# Autodesk Inventor assembly: _VK_Indexier-Station
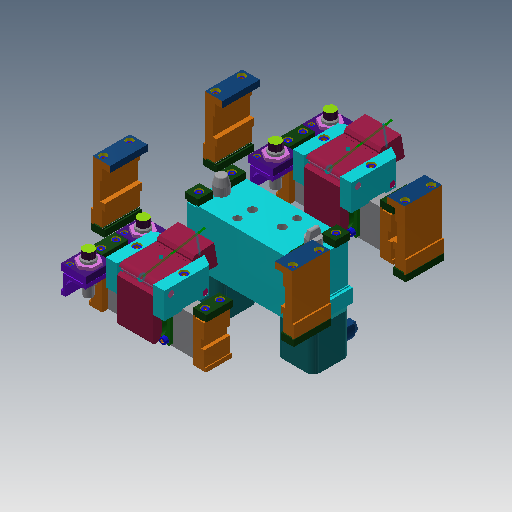
[picture p0: Inventor's stored thumbnail of the model, 512x512]
Saved by Autodesk Inventor 2019 (Build 230136000, 136)
## iProperties
Created: 2023-11-18
Part Number: _VK_Indexier-Station
Material: Generisch
Document SubType Name: Assembly
Designer: RP
Author: RP
## Documents named in this file (4)
- C:\Users\RP\Documents\Inventor\Projekt_Angelspule\_Verkettung\_VK_Indexier-Station.iam
- C:\Users\RP\Documents\Inventor\Projekt_Angelspule\_Verkettung\__VK_Stopper_Vor-Stopper_Einheit.iam
- C:\Users\RP\Documents\Inventor\Projekt_Angelspule\_Verkettung\__VK_Indexierung.iam
- C:\Users\RP\Documents\Inventor\Projekt_Angelspule\_Verkettung\__VK_Niederhalter.ipt
## Components (6 placed, 3 different names)
1. __VK_Stopper_Vor-Stopper_Einheit:1 [sub-assembly]
2. __VK_Indexierung:1 [sub-assembly] — Fluchtend:3, Fluchtend:4, Fluchtend:10
3. __VK_Niederhalter:1 — Fluchtend:20, Fluchtend:21
4. __VK_Niederhalter:2 — Fluchtend:21
5. __VK_Niederhalter:3
6. __VK_Niederhalter:4
## Relationships (17: Flush 14, Mate 3)
- Fluchtend:3 [Flush]: __VK_Indexierung:1
- Fluchtend:4 [Flush]: __VK_Indexierung:1
- Fluchtend:10 [Flush]: __VK_Indexierung:1
- [Flush]: __VK_Niederhalter:1 ↔ __VK_Niederhalter:3
- [Flush]: __VK_Niederhalter:1 ↔ __VK_Niederhalter:3
- [Flush]: __VK_Niederhalter:2 ↔ __VK_Niederhalter:4
- [Flush]: __VK_Niederhalter:2 ↔ __VK_Niederhalter:4
- [Mate] (127.1 mm): __VK_Niederhalter:1
- [Mate] (127.1 mm): __VK_Niederhalter:3
- [Flush] (127.1 mm): __VK_Niederhalter:4
- [Flush] (127.1 mm): __VK_Niederhalter:2
- [Flush]: __VK_Niederhalter:3 ↔ __VK_Niederhalter:4
- [Flush]: __VK_Niederhalter:1 ↔ __VK_Niederhalter:2
- [Flush] (100 mm): __VK_Niederhalter:3
- [Mate] (-100 mm): __VK_Niederhalter:1
- Fluchtend:20 [Flush] (29.415 mm): __VK_Niederhalter:1
- Fluchtend:21 [Flush]: __VK_Niederhalter:1 ↔ __VK_Niederhalter:2
